# Autodesk Inventor assembly: HCMUTE-CDT23-FRAME_ASEMBLY
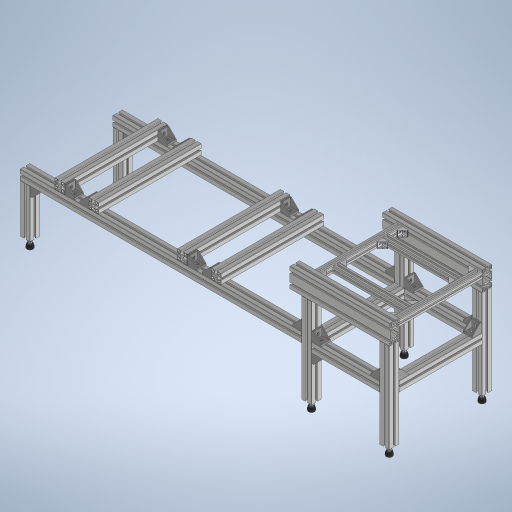
[picture p0: Inventor's stored thumbnail of the model, 512x512]
Saved by Autodesk Inventor 2023 (Build 270158000, 158)
## iProperties
_SolveAssemblyDoc: Frame Generator Solve Assembly
_Version: 25.0.0
Created: 2023-11-19
Part Number: HCMUTE-CDT23-FRAME_ASEMBLY
Document SubType Name: Assembly
Designer: havie
Mass: 3541.1 g
Surface Area: 24843.7 cm^2
Volume: 2332.81 cm^3
Density: 1.51795 g/cm^3
Author: havie
## Documents named in this file (6)
- D:\DO_AN_CDT\1.1. PART\HCMUTE-CDT23-FRAME_ASEMBLY.iam
- D:\DO_AN_CDT\1.1. PART\HCMUTE-CDT23-SKETCH_FRAME.ipt
- D:\DO_AN_CDT\1.1. PART\HCMUTE-CDT23-FRAME_ASEMBLY\Frame\Frame 1700330515848.iam
- C:\Users\havie\Documents\Inventor\Content Center Files\R2023\en-US\302828\302828.ipt
- C:\Users\havie\Documents\Inventor\Content Center Files\R2023\en-US\301818\301818.ipt
- C:\Users\havie\Documents\Inventor\Content Center Files\R2023\en-US\402005\402005.ipt
## Components (38 placed, 5 different names)
1. HCMUTE-CDT23-SKETCH_FRAME:1
2. Frame 1700330515848:1 [sub-assembly] — Mate:1, Mate:2, Flush:1, Mate:3, Mate:4, Flush:2, Mate:5, Mate:7, Mate:8, Flush:4, Mate:9, Mate:11, Mate:12, Flush:6, Mate:13, Mate:14, Flush:7, Mate:15, Mate:16, Flush:8, Mate:17, Mate:18, Flush:9, Mate:19, Mate:20, Flush:10, Mate:21, Mate:22, Flush:11, Mate:23, Flush:12, Mate:24, Mate:25, Mate:26, Flush:13, Mate:27, Mate:28, Flush:14, Mate:29, Mate:30, Flush:15, Mate:31, Mate:32, Mate:33, Mate:34, Mate:35, Mate:36, Mate:37, Mate:38, Mate:39, Mate:40, Mate:41, Flush:17, Mate:42, Mate:43, Mate:44, Mate:45, Mate:46, Mate:47
3. 302828 302828:1 — Mate:1, Mate:2, Flush:1
4. 302828 302828:2 — Mate:3, Mate:4, Flush:2, Flush:20
5. 302828 302828:3 — Mate:5, Mate:45, Flush:20
6. 302828 302828:4 — Mate:7, Mate:8, Flush:4, Flush:18
7. 302828 302828:5 — Mate:13, Mate:14, Flush:7
8. 302828 302828:6 — Mate:15, Mate:16, Flush:8
9. 302828 302828:7 — Mate:9, Mate:42, Flush:18
10. 302828 302828:8 — Mate:11, Mate:12, Flush:6
11. 302828 302828:9 — Mate:17, Mate:18, Flush:9
12. 302828 302828:10 — Mate:19, Mate:20, Flush:10
13. 302828 302828:11 — Mate:21, Mate:22, Flush:11
14. 301818 302828.1:1 — Mate:27, Mate:28, Flush:14
15. 301818 302828.1:2 — Mate:23, Flush:12, Mate:24
16. 301818 302828.1:3 — Mate:25, Mate:26, Flush:13
17. 301818 302828.1:4 — Mate:29, Mate:30, Flush:15
18. 402005 402005:1 — Mate:31, Mate:32, Flush:16
19. 402005 402005:2 — Mate:33, Flush:16
20. 402005 402005:3 — Mate:34, Mate:35
21. 402005 402005:4 — Mate:36, Mate:37
22. 402005 402005:5 — Mate:40, Mate:41
23. 402005 402005:6 — Mate:38, Mate:39
24. 302828 302828:12
25. 302828 302828:13 — Flush:21
26. 302828 302828:15 — Flush:19
27. 302828 302828:16
28. 302828 302828:17
29. 302828 302828:19
30. 302828 302828:21
31. 302828 302828:22
32. 302828 302828:23
33. 301818 302828.1:5
34. 301818 302828.1:6
35. 301818 302828.1:7
36. 301818 302828.1:8
37. 302828 302828:24 — Mate:43, Mate:44, Flush:19
38. 302828 302828:25 — Mate:46, Mate:47, Flush:21
## Relationships (64: Mate 45, Flush 19)
- Mate:1: Frame 1700330515848:1 ↔ 302828 302828:1
- Mate:2: Frame 1700330515848:1 ↔ 302828 302828:1
- Flush:1 (1 mm): Frame 1700330515848:1 ↔ 302828 302828:1
- Mate:3: Frame 1700330515848:1 ↔ 302828 302828:2
- Mate:4: Frame 1700330515848:1 ↔ 302828 302828:2
- Flush:2 (1 mm): Frame 1700330515848:1 ↔ 302828 302828:2
- Mate:5: Frame 1700330515848:1 ↔ 302828 302828:3
- Mate:7: Frame 1700330515848:1 ↔ 302828 302828:4
- Mate:8: Frame 1700330515848:1 ↔ 302828 302828:4
- Flush:4 (1 mm): Frame 1700330515848:1 ↔ 302828 302828:4
- Mate:9: Frame 1700330515848:1 ↔ 302828 302828:7
- Mate:11: Frame 1700330515848:1 ↔ 302828 302828:8
- Mate:12: Frame 1700330515848:1 ↔ 302828 302828:8
- Flush:6 (1 mm): Frame 1700330515848:1 ↔ 302828 302828:8
- Mate:13: Frame 1700330515848:1 ↔ 302828 302828:5
- Mate:14: Frame 1700330515848:1 ↔ 302828 302828:5
- Flush:7 (1 mm): Frame 1700330515848:1 ↔ 302828 302828:5
- Mate:15: Frame 1700330515848:1 ↔ 302828 302828:6
- Mate:16: Frame 1700330515848:1 ↔ 302828 302828:6
- Flush:8 (1 mm): Frame 1700330515848:1 ↔ 302828 302828:6
- Mate:17: Frame 1700330515848:1 ↔ 302828 302828:9
- Mate:18: Frame 1700330515848:1 ↔ 302828 302828:9
- Flush:9 (1 mm): Frame 1700330515848:1 ↔ 302828 302828:9
- Mate:19: Frame 1700330515848:1 ↔ 302828 302828:10
- Mate:20: Frame 1700330515848:1 ↔ 302828 302828:10
- Flush:10 (1 mm): Frame 1700330515848:1 ↔ 302828 302828:10
- Mate:21: Frame 1700330515848:1 ↔ 302828 302828:11
- Mate:22: Frame 1700330515848:1 ↔ 302828 302828:11
- Flush:11 (1 mm): Frame 1700330515848:1 ↔ 302828 302828:11
- Mate:23: Frame 1700330515848:1 ↔ 301818 302828.1:2
- Flush:12 (1 mm): Frame 1700330515848:1 ↔ 301818 302828.1:2
- Mate:24: Frame 1700330515848:1 ↔ 301818 302828.1:2
- Mate:25: Frame 1700330515848:1 ↔ 301818 302828.1:3
- Mate:26: Frame 1700330515848:1 ↔ 301818 302828.1:3
- Flush:13 (1 mm): Frame 1700330515848:1 ↔ 301818 302828.1:3
- Mate:27: Frame 1700330515848:1 ↔ 301818 302828.1:1
- Mate:28: Frame 1700330515848:1 ↔ 301818 302828.1:1
- Flush:14 (1 mm): Frame 1700330515848:1 ↔ 301818 302828.1:1
- Mate:29: Frame 1700330515848:1 ↔ 301818 302828.1:4
- Mate:30: Frame 1700330515848:1 ↔ 301818 302828.1:4
- Flush:15 (1 mm): Frame 1700330515848:1 ↔ 301818 302828.1:4
- Mate:31: Frame 1700330515848:1 ↔ 402005 402005:1
- Mate:32 (1.5 mm): Frame 1700330515848:1 ↔ 402005 402005:1
- Mate:33: Frame 1700330515848:1 ↔ 402005 402005:2
- Flush:16: 402005 402005:1 ↔ 402005 402005:2
- Mate:34: Frame 1700330515848:1 ↔ 402005 402005:3
- Mate:35: Frame 1700330515848:1 ↔ 402005 402005:3
- Mate:36: Frame 1700330515848:1 ↔ 402005 402005:4
- Mate:37: Frame 1700330515848:1 ↔ 402005 402005:4
- Mate:38: Frame 1700330515848:1 ↔ 402005 402005:6
- Mate:39: Frame 1700330515848:1 ↔ 402005 402005:6
- Mate:40: Frame 1700330515848:1 ↔ 402005 402005:5
- Mate:41: Frame 1700330515848:1 ↔ 402005 402005:5
- Flush:17 (-155 mm): Frame 1700330515848:1
- Mate:42: Frame 1700330515848:1 ↔ 302828 302828:7
- Flush:18: 302828 302828:4 ↔ 302828 302828:7
- Mate:43: Frame 1700330515848:1 ↔ 302828 302828:24
- Mate:44: Frame 1700330515848:1 ↔ 302828 302828:24
- Flush:19: 302828 302828:15 ↔ 302828 302828:24
- Mate:45: Frame 1700330515848:1 ↔ 302828 302828:3
- Flush:20: 302828 302828:2 ↔ 302828 302828:3
- Mate:46: Frame 1700330515848:1 ↔ 302828 302828:25
- Mate:47: Frame 1700330515848:1 ↔ 302828 302828:25
- Flush:21: 302828 302828:13 ↔ 302828 302828:25
